# Autodesk Inventor assembly: CLB_055_ScissorBarWithSpacer
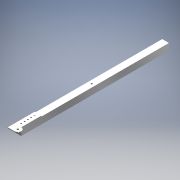
[picture p0: Inventor's stored thumbnail of the model, 180x180]
Saved by Autodesk Inventor 2018.3 (Build 223284000, 284)
## iProperties
Created: 2020-02-16
Part Number: CLB_055_ScissorBarWithSpacer
Document SubType Name: Assembly
Designer: 22perngrac
Author: 22perngrac
## Documents named in this file (4)
- C:\Users\22perngrac\Documents\GrabCAD\Infinite Recharge 2020\Build season\CLB_055_ScissorBarBottomWithPlug.iam
- C:\Users\22perngrac\Documents\GrabCAD\Infinite Recharge 2020\Build season\CLB_052_ScissorLiftPlug.ipt
- C:\Users\22perngrac\Documents\GrabCAD\Infinite Recharge 2020\Build season\CLB_029_ScissorLiftBarBottom.ipt
- C:\Users\22perngrac\Documents\GrabCAD\Infinite Recharge 2020\Build season\CLB_027_LifterBracket.ipt
## Components (4 placed, 3 different names)
1. CLB_052_ScissorLiftPlug:1 — Mate:1, Mate:2, Flush:3
2. CLB_052_ScissorLiftPlug:2 — Mate:3, Mate:4, Flush:2
3. CLB_029_ScissorLiftBarBottom:1 — Mate:1, Mate:2, Mate:3, Mate:4, Flush:2, Flush:3, Mate:5, Flush:4, Flush:5
4. CLB_027_LifterBracket:1 — Mate:5, Flush:4, Flush:5
## Relationships (9: Mate 5, Flush 4)
- Mate:1: CLB_052_ScissorLiftPlug:1 ↔ CLB_029_ScissorLiftBarBottom:1
- Mate:2: CLB_052_ScissorLiftPlug:1 ↔ CLB_029_ScissorLiftBarBottom:1
- Mate:3: CLB_052_ScissorLiftPlug:2 ↔ CLB_029_ScissorLiftBarBottom:1
- Mate:4: CLB_052_ScissorLiftPlug:2 ↔ CLB_029_ScissorLiftBarBottom:1
- Flush:2: CLB_052_ScissorLiftPlug:2 ↔ CLB_029_ScissorLiftBarBottom:1
- Flush:3: CLB_052_ScissorLiftPlug:1 ↔ CLB_029_ScissorLiftBarBottom:1
- Mate:5: CLB_029_ScissorLiftBarBottom:1 ↔ CLB_027_LifterBracket:1
- Flush:4: CLB_029_ScissorLiftBarBottom:1 ↔ CLB_027_LifterBracket:1
- Flush:5 (-25.4 mm): CLB_029_ScissorLiftBarBottom:1 ↔ CLB_027_LifterBracket:1
